# Autodesk Inventor assembly: frame
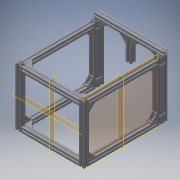
[picture p0: Inventor's stored thumbnail of the model, 180x180]
Saved by Autodesk Inventor 2019.3 (Build 233278000, 278)
## iProperties
Created: 2019-04-14
Part Number: frame
Document SubType Name: Assembly
Designer: peter
Author: peter
## Documents named in this file (25)
- C:\Users\peter\OneDrive\Documents\Inventor\Automated Bar\frame.iam
- C:\Users\peter\OneDrive\Documents\Inventor\Automated Bar\extrusion_250.ipt
- C:\Users\peter\OneDrive\Documents\Inventor\Automated Bar\extrusion_300.ipt
- C:\Users\peter\OneDrive\Documents\Inventor\Automated Bar\bracket.ipt
- C:\Users\peter\OneDrive\Documents\Inventor\Automated Bar\bracket_MIR.ipt
- C:\Users\peter\OneDrive\Documents\Inventor\Automated Bar\bracket_MIR1.ipt
- C:\Users\peter\OneDrive\Documents\Inventor\Automated Bar\bracket_MIR_MIR.ipt
- C:\Users\peter\OneDrive\Documents\Inventor\Automated Bar\bracket_MIR2.ipt
- C:\Users\peter\OneDrive\Documents\Inventor\Automated Bar\bracket_MIR_MIR1.ipt
- C:\Users\peter\OneDrive\Documents\Inventor\Automated Bar\bracket_MIR1_MIR.ipt
- C:\Users\peter\OneDrive\Documents\Inventor\Automated Bar\bracket_MIR_MIR_MIR.ipt
- C:\Users\peter\OneDrive\Documents\Inventor\Automated Bar\bracket_MIR3.ipt
- C:\Users\peter\OneDrive\Documents\Inventor\Automated Bar\extrusion_95.ipt
- C:\Users\peter\OneDrive\Documents\Inventor\Automated Bar\bracket_MIR4.ipt
- C:\Users\peter\OneDrive\Documents\Inventor\Automated Bar\clip3.ipt
- C:\Users\peter\OneDrive\Documents\Inventor\Automated Bar\clip3_MIR.ipt
- C:\Users\peter\OneDrive\Documents\Inventor\Automated Bar\clip3_MIR1.ipt
- C:\Users\peter\OneDrive\Documents\Inventor\Automated Bar\clip3_MIR_MIR.ipt
- C:\Users\peter\OneDrive\Documents\Inventor\Automated Bar\clip3_MIR2.ipt
- C:\Users\peter\OneDrive\Documents\Inventor\Automated Bar\clip3_MIR_MIR1.ipt
- C:\Users\peter\OneDrive\Documents\Inventor\Automated Bar\clip3_MIR1_MIR.ipt
- C:\Users\peter\OneDrive\Documents\Inventor\Automated Bar\clip3_MIR_MIR_MIR.ipt
- C:\Users\peter\OneDrive\Documents\Inventor\Automated Bar\bracket_MIR5.ipt
- C:\Users\peter\OneDrive\Documents\Inventor\Automated Bar\bracket_MIR6.ipt
- C:\Users\peter\OneDrive\Documents\Inventor\Automated Bar\bracket_MIR5_MIR.ipt
## Components (38 placed, 24 different names)
1. extrusion_250:1 — Mate:1, Flush:1, Flush:2, Mate:3, Mate:4, Flush:5
2. extrusion_250:2 — Mate:1, Flush:1, Flush:2, Mate:6, Flush:8, Flush:9, Flush:10, Flush:11, Mate:7, Mate:17
3. extrusion_250:3 — Mate:5, Flush:6, Flush:7, Mate:22, Mate:23
4. extrusion_250:4 — Mate:8, Flush:12, Flush:13, Mate:9, Flush:14, Flush:15, Symmetry:2, Flush:28
5. extrusion_300:1 — Mate:3, Mate:4, Flush:5, Mate:5, Flush:6, Flush:7, Mate:16, Flush:25, Mate:18, Flush:26, Mate:20
6. extrusion_300:2 — Flush:10, Flush:11, Mate:7, Flush:23, Mate:15
7. extrusion_300:3 — Mate:8, Flush:12, Flush:13, Symmetry:4
8. extrusion_300:4 — Mate:9, Flush:14, Flush:15, Mate:10, Flush:16, Flush:17, Symmetry:4
9. extrusion_300:5 — Mate:6, Flush:8, Flush:9, Flush:18, Flush:19, Mate:11, Mate:25
10. extrusion_250:5 — Mate:10, Flush:16, Flush:17, Flush:20, Flush:22, Symmetry:2, Symmetry:3
11. extrusion_250:6 — Flush:18, Flush:19, Mate:11, Mate:12, Flush:21, Mate:13, Mate:14, Flush:24, Symmetry:1, Symmetry:3
12. extrusion_250:7 — Flush:22, Flush:23, Mate:13
13. extrusion_250:8 — Flush:20, Mate:12, Flush:21, Symmetry:1, Mate:24, Flush:29
14. bracket:3 — Mate:14, Mate:15, Flush:24
15. bracket_MIR:1
16. bracket_MIR1:1
17. bracket_MIR_MIR:1
18. bracket_MIR2:1
19. bracket_MIR_MIR1:1
20. bracket_MIR1_MIR:1
21. bracket_MIR_MIR_MIR:1
22. bracket:4 — Mate:16, Mate:17, Flush:25
23. bracket_MIR3:1
24. extrusion_95:1 — Mate:18, Mate:19, Flush:26, Mate:21, Flush:27
25. bracket:5 — Mate:20, Mate:21, Flush:27
26. bracket_MIR4:1
27. clip3:1 — Mate:22, Mate:23, Flush:28
28. clip3_MIR:1
29. clip3_MIR1:1
30. clip3_MIR_MIR:1
31. clip3_MIR2:1
32. clip3_MIR_MIR1:1
33. clip3_MIR1_MIR:1
34. clip3_MIR_MIR_MIR:1
35. bracket:6 — Mate:24, Mate:25, Flush:29
36. bracket_MIR5:1
37. bracket_MIR6:1
38. bracket_MIR5_MIR:1
## Relationships (58: Flush 29, Mate 25, Symmetry 4)
- Mate:1: extrusion_250:1 ↔ extrusion_250:2
- Flush:1: extrusion_250:1 ↔ extrusion_250:2
- Flush:2: extrusion_250:1 ↔ extrusion_250:2
- [Mate]: extrusion_250:3 ↔ extrusion_250:4
- [Flush]: extrusion_250:3 ↔ extrusion_250:4
- [Flush]: extrusion_250:3 ↔ extrusion_250:4
- Mate:3: extrusion_250:1 ↔ extrusion_300:1
- Mate:4: extrusion_250:1 ↔ extrusion_300:1
- Flush:5: extrusion_250:1 ↔ extrusion_300:1
- Mate:5: extrusion_250:3 ↔ extrusion_300:1
- Flush:6: extrusion_250:3 ↔ extrusion_300:1
- Flush:7: extrusion_250:3 ↔ extrusion_300:1
- Mate:6: extrusion_250:2 ↔ extrusion_300:5
- Flush:8: extrusion_250:2 ↔ extrusion_300:5
- Flush:9: extrusion_250:2 ↔ extrusion_300:5
- Flush:10: extrusion_250:2 ↔ extrusion_300:2
- Flush:11: extrusion_250:2 ↔ extrusion_300:2
- Mate:7: extrusion_250:2 ↔ extrusion_300:2
- Mate:8: extrusion_250:4 ↔ extrusion_300:3
- Flush:12: extrusion_250:4 ↔ extrusion_300:3
- Flush:13: extrusion_250:4 ↔ extrusion_300:3
- Mate:9: extrusion_250:4 ↔ extrusion_300:4
- Flush:14: extrusion_250:4 ↔ extrusion_300:4
- Flush:15: extrusion_250:4 ↔ extrusion_300:4
- Mate:10: extrusion_300:4 ↔ extrusion_250:5
- Flush:16: extrusion_300:4 ↔ extrusion_250:5
- Flush:17: extrusion_300:4 ↔ extrusion_250:5
- Flush:18: extrusion_300:5 ↔ extrusion_250:6
- Flush:19: extrusion_300:5 ↔ extrusion_250:6
- Mate:11: extrusion_300:5 ↔ extrusion_250:6
- Flush:20: extrusion_250:5 ↔ extrusion_250:8
- Mate:12 (3 mm): extrusion_250:6 ↔ extrusion_250:8
- Flush:21: extrusion_250:6 ↔ extrusion_250:8
- Flush:22: extrusion_250:5 ↔ extrusion_250:7
- Flush:23: extrusion_300:2 ↔ extrusion_250:7
- Mate:13 (3 mm): extrusion_250:6 ↔ extrusion_250:7
- Mate:14: extrusion_250:6 ↔ bracket:3
- Mate:15: extrusion_300:2 ↔ bracket:3
- Flush:24 (1 mm): extrusion_250:6 ↔ bracket:3
- Symmetry:1: extrusion_250:6 ↔ extrusion_250:8
- Symmetry:2: extrusion_250:4 ↔ extrusion_250:5
- Symmetry:3: extrusion_250:5 ↔ extrusion_250:6
- Mate:16: extrusion_300:1 ↔ bracket:4
- Mate:17: extrusion_250:2 ↔ bracket:4
- Flush:25 (1 mm): extrusion_300:1 ↔ bracket:4
- Mate:18: extrusion_300:1 ↔ extrusion_95:1
- Mate:19: extrusion_95:1
- Flush:26: extrusion_300:1 ↔ extrusion_95:1
- Mate:20: extrusion_300:1 ↔ bracket:5
- Mate:21: extrusion_95:1 ↔ bracket:5
- Flush:27 (1 mm): extrusion_95:1 ↔ bracket:5
- Mate:22: extrusion_250:3 ↔ clip3:1
- Mate:23: extrusion_250:3 ↔ clip3:1
- Flush:28 (25 mm): extrusion_250:4 ↔ clip3:1
- Symmetry:4: extrusion_300:3 ↔ extrusion_300:4
- Mate:24: extrusion_250:8 ↔ bracket:6
- Mate:25: extrusion_300:5 ↔ bracket:6
- Flush:29 (1 mm): extrusion_250:8 ↔ bracket:6
## Named parameters: d3_d0 = 0 mm, d4_d1 = 0 mm, d5_d2 = 0 mm
